# Autodesk Inventor assembly: Arm
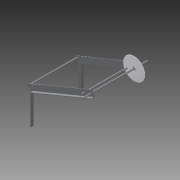
[picture p0: Inventor's stored thumbnail of the model, 180x180]
Saved by Autodesk Inventor 2013 (Build 170138000, 138)
## iProperties
Created: 2014-01-18
Part Number: Arm
Document SubType Name: Assembly
Designer: 272817
Author: 272817
## Documents named in this file (8)
- E:\Robotics\FRC\2014\CAD\Robot\Catapult\ArmOld.iam
- E:\Robotics\FRC\2014\CAD\Robot\Catapult\Arm\CatapultArmOld-Left.ipt
- E:\Robotics\FRC\2014\CAD\Robot\Catapult\Arm\CatapultArmOld-Right.ipt
- E:\Robotics\FRC\2014\CAD\Robot\Catapult\Arm\CatapultSprocket.ipt
- E:\Robotics\FRC\2014\CAD\Robot\Catapult\Arm\CatapultAxle.ipt
- E:\Robotics\FRC\2014\CAD\Robot\Catapult\Arm\CatapultAxleSupport.ipt
- E:\Robotics\FRC\2014\CAD\Robot\Catapult\Arm\CrossBrace.ipt
- E:\Robotics\FRC\2014\CAD\Robot\Catapult\Arm\BarHolder.ipt
## Components (8 placed, 7 different names)
1. CatapultArmOld-Left:1 — Flush:1, Flush:2, Mate:1, Mate:2, Mate:3, Flush:4, Flush:5, Mate:14, Flush:7
2. CatapultArmOld-Right:1 — Flush:1, Flush:2, Flush:3, Mate:9, Flush:6, Mate:10
3. CatapultSprocket:1 — Mate:3, Mate:4, Mate:5
4. CatapultAxle:1 — Mate:1, Mate:4, Flush:5
5. CatapultAxleSupport:1 — Mate:2, Mate:5, Flush:3, Flush:4
6. CrossBrace:1 — Mate:11, Mate:12, Mate:13
7. BarHolder:1 — Mate:9, Flush:6, Mate:10, Mate:11, Mate:12
8. BarHolder:2 — Mate:13, Mate:14, Flush:7
## Relationships (18: Mate 11, Flush 7)
- Flush:1: CatapultArmOld-Left:1 ↔ CatapultArmOld-Right:1
- Flush:2: CatapultArmOld-Left:1 ↔ CatapultArmOld-Right:1
- Mate:1: CatapultArmOld-Left:1 ↔ CatapultAxle:1
- Mate:2: CatapultArmOld-Left:1 ↔ CatapultAxleSupport:1
- Mate:3 (38.1 mm): CatapultArmOld-Left:1 ↔ CatapultSprocket:1
- Mate:4: CatapultSprocket:1 ↔ CatapultAxle:1
- Mate:5: CatapultSprocket:1 ↔ CatapultAxleSupport:1
- Flush:3: CatapultArmOld-Right:1 ↔ CatapultAxleSupport:1
- Flush:4: CatapultArmOld-Left:1 ↔ CatapultAxleSupport:1
- Flush:5 (-69.85 mm): CatapultArmOld-Left:1 ↔ CatapultAxle:1
- Mate:9: CatapultArmOld-Right:1 ↔ BarHolder:1
- Flush:6: CatapultArmOld-Right:1 ↔ BarHolder:1
- Mate:10: CatapultArmOld-Right:1 ↔ BarHolder:1
- Mate:11: CrossBrace:1 ↔ BarHolder:1
- Mate:12: CrossBrace:1 ↔ BarHolder:1
- Mate:13: CrossBrace:1 ↔ BarHolder:2
- Mate:14: CatapultArmOld-Left:1 ↔ BarHolder:2
- Flush:7: CatapultArmOld-Left:1 ↔ BarHolder:2
